# Autodesk Inventor assembly: base assembly(1)
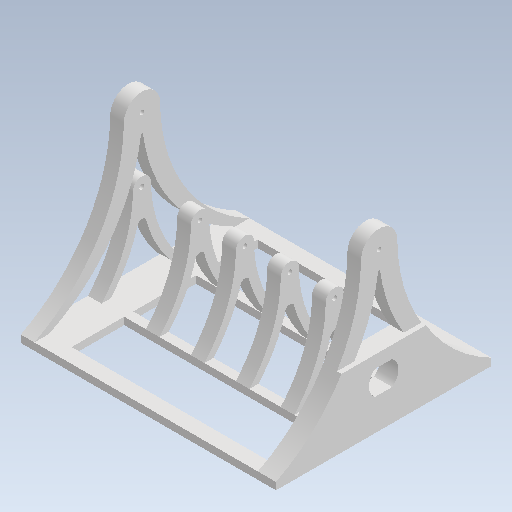
[picture p0: Inventor's stored thumbnail of the model, 512x512]
Saved by Autodesk Inventor 2023 (Build 270158000, 158)
## iProperties
Created: 2023-03-30
Part Number: base assembly(1)
Document SubType Name: Assembly
Designer: dverd
Author: dverd
## Documents named in this file (4)
- C:\Users\dverd\OneDrive\Documents\ME\ME 354\turbine lab 2.0\CAD\base assembly(1).iam
- C:\Users\dverd\OneDrive\Documents\ME\ME 354\turbine lab 2.0\CAD\base plate wo supports.iam
- C:\Users\dverd\OneDrive\Documents\ME\ME 354\turbine lab 2.0\CAD\transfer gear rod support(4).ipt
- C:\Users\dverd\OneDrive\Documents\ME\ME 354\turbine lab 2.0\CAD\transfer gear rod support end(1).ipt
## Components (6 placed, 3 different names)
1. base plate wo supports:1 [sub-assembly] — Angle:1, Mate:4, Mate:5, Mate:6, Mate:7, Flush:4, Mate:9, Flush:5
2. transfer gear rod support(4):1 — Mate:1, Flush:3, Mate:7, Mate:8
3. transfer gear rod support(4):2 — Mate:1, Mate:2, Flush:2, Flush:3, Mate:4
4. transfer gear rod support(4):3 — Mate:2, Mate:3, Flush:1, Flush:2, Mate:5
5. transfer gear rod support(4):4 — Mate:3, Flush:1, Angle:1, Mate:6, Flush:5
6. transfer gear rod support end(1):1 — Mate:8, Flush:4, Mate:9
## Relationships (15: Mate 9, Flush 5, Angle 1)
- Mate:1: transfer gear rod support(4):1 ↔ transfer gear rod support(4):2
- Mate:2: transfer gear rod support(4):2 ↔ transfer gear rod support(4):3
- Mate:3: transfer gear rod support(4):3 ↔ transfer gear rod support(4):4
- Flush:1 (31.4452 mm): transfer gear rod support(4):3 ↔ transfer gear rod support(4):4
- Flush:2 (31.4452 mm): transfer gear rod support(4):2 ↔ transfer gear rod support(4):3
- Flush:3 (31.4452 mm): transfer gear rod support(4):1 ↔ transfer gear rod support(4):2
- Angle:1 (0 deg): base plate wo supports:1 ↔ transfer gear rod support(4):4
- Mate:4: base plate wo supports:1 ↔ transfer gear rod support(4):2
- Mate:5: base plate wo supports:1 ↔ transfer gear rod support(4):3
- Mate:6: base plate wo supports:1 ↔ transfer gear rod support(4):4
- Mate:7: base plate wo supports:1 ↔ transfer gear rod support(4):1
- Mate:8: transfer gear rod support(4):1 ↔ transfer gear rod support end(1):1
- Flush:4: base plate wo supports:1 ↔ transfer gear rod support end(1):1
- Mate:9: base plate wo supports:1 ↔ transfer gear rod support end(1):1
- Flush:5 (34.2392 mm): base plate wo supports:1 ↔ transfer gear rod support(4):4
